# Autodesk Inventor assembly: Assembly2
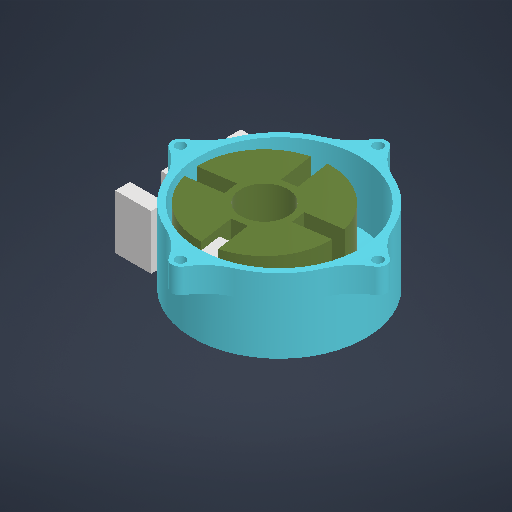
[picture p0: Inventor's stored thumbnail of the model, 512x512]
Saved by Autodesk Inventor 2025.3 (Build 293356000, 356)
## iProperties
Created: 2025-10-20
Part Number: Assembly2
Document SubType Name: Assembly
Designer: sophi
Author: sophi
## Documents named in this file (5)
- C:\Users\sophi\OneDrive - Universidad de los andes\Documentos\1 Universidad\5 Semestre\Herramientas\Huron-Hudson\Vane Engine\Vane V3\Assembly2.iam
- C:\Users\sophi\OneDrive - Universidad de los andes\Documentos\1 Universidad\5 Semestre\Herramientas\Huron-Hudson\Vane Engine\Vane V3\carcaza.ipt
- C:\Users\sophi\OneDrive - Universidad de los andes\Documentos\1 Universidad\5 Semestre\Herramientas\Huron-Hudson\Vane Engine\Vane V3\rotor.ipt
- C:\Users\sophi\OneDrive - Universidad de los andes\Documentos\1 Universidad\5 Semestre\Herramientas\Huron-Hudson\Vane Engine\Vane V3\tapa.ipt
- C:\Users\sophi\OneDrive - Universidad de los andes\Documentos\1 Universidad\5 Semestre\Herramientas\Huron-Hudson\Vane Engine\Vane V3\paletas.ipt
## Components (7 placed, 4 different names)
1. carcaza:1 — Flush:1, Flush:2, Flush:3, Mate:2
2. rotor:1 — Mate:2
3. tapa:1
4. paletas:1
5. paletas:2
6. paletas:3 — Flush:5
7. paletas:4
## Relationships (6: Flush 5, Mate 1)
- Flush:1: carcaza:1
- Flush:2: carcaza:1
- Flush:3: carcaza:1
- Flush:5 (-3 mm): paletas:3
- Flush:6
- Mate:2: carcaza:1 ↔ rotor:1
